# Autodesk Inventor assembly: Z-axis Left Plate
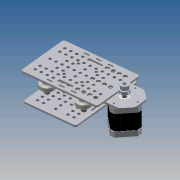
[picture p0: Inventor's stored thumbnail of the model, 180x180]
Saved by Autodesk Inventor 2016 (Build 200138000, 138)
## iProperties
Created: 2015-10-03
Part Number: Z-axis Left Plate
Document SubType Name: Assembly
Designer: Solomon
Author: Solomon
## Documents named in this file (7)
- C:\Users\Solomon\Documents\Inventor\jonathan-printer\Z-axis Right.iam
- C:\Users\Solomon\Documents\Inventor\jonathan-printer\V Slot Part Files\V Slot Plates\Large Build Plate.ipt
- C:\Users\Solomon\Documents\Inventor\jonathan-printer\V Slot Part Files\assembledwheel.iam
- C:\Users\Solomon\Documents\Inventor\jonathan-printer\M1173041- NEMA 17.ipt
- C:\Users\Solomon\Documents\Inventor\jonathan-printer\V Slot Part Files\V Slot Plates\Threaded Rod Plate.ipt
- C:\Users\Solomon\Documents\Inventor\jonathan-printer\Imported Components\GT2_20tooth\GT2_20tooth.ipt
- C:\Users\Solomon\Documents\Inventor\jonathan-printer\V Slot Part Files\V Slot Plates\Metric 8mm ACME Block.ipt
## Components (11 placed, 6 different names)
1. assembledwheel:1 [sub-assembly] — Angle:8, Mate:15, Mate:20, Angle:16
2. assembledwheel:2 [sub-assembly] — Angle:8, Mate:18, Mate:19, Angle:16, Angle:17
3. assembledwheel:3 [sub-assembly] — Angle:9, Mate:14, Mate:16, Mate:17, Angle:17, Angle:18, Angle:20
4. assembledwheel:4 [sub-assembly] — Mate:6, Mate:21, Mate:22, Angle:18, Angle:19
5. Large Build Plate:2 — Mate:6, Angle:9, Angle:14, Angle:15, Mate:16, Mate:17, Mate:18, Mate:20, Mate:21, Angle:21, Angle:22, Mate:23
6. M1173041- NEMA 17:1 — Mate:24, Angle:23, Angle:24, Insert:1
7. Large Build Plate:3 — Angle:14, Angle:15, Mate:14, Mate:15, Mate:19, Mate:22, Angle:19, Angle:20, Angle:26, Angle:27, Angle:28, Angle:29, Mate:25, Mate:26
8. Threaded Rod Plate:1 — Angle:21, Angle:22, Mate:23, Mate:24, Angle:23, Angle:24, Angle:25
9. GT2_20tooth:1 — Angle:25, Insert:1
10. Metric 8mm ACME Block:1 — Angle:26, Angle:27, Angle:28, Angle:29, Mate:25, Flush:1, Flush:2, Angle:30, Angle:31, Angle:32
11. Metric 8mm ACME Block:2 — Flush:1, Flush:2, Angle:30, Angle:31, Angle:32, Mate:26
## Relationships (38: Angle 21, Mate 14, Flush 2, Insert 1)
- Mate:6: assembledwheel:4 ↔ Large Build Plate:2
- Angle:8 (0 deg): assembledwheel:1 ↔ assembledwheel:2
- Angle:9 (0 deg): assembledwheel:3 ↔ Large Build Plate:2
- Angle:14 (0 deg): Large Build Plate:2 ↔ Large Build Plate:3
- Angle:15 (0 deg): Large Build Plate:2 ↔ Large Build Plate:3
- Mate:14: assembledwheel:3 ↔ Large Build Plate:3
- Mate:15: assembledwheel:1 ↔ Large Build Plate:3
- Mate:16: assembledwheel:3 ↔ Large Build Plate:2
- Mate:17: assembledwheel:3 ↔ Large Build Plate:2
- Mate:18: assembledwheel:2 ↔ Large Build Plate:2
- Mate:19: assembledwheel:2 ↔ Large Build Plate:3
- Mate:20: assembledwheel:1 ↔ Large Build Plate:2
- Angle:16 (0 deg): assembledwheel:1 ↔ assembledwheel:2
- Angle:17 (0 deg): assembledwheel:2 ↔ assembledwheel:3
- Mate:21: assembledwheel:4 ↔ Large Build Plate:2
- Mate:22: assembledwheel:4 ↔ Large Build Plate:3
- Angle:18 (0 deg): assembledwheel:3 ↔ assembledwheel:4
- Angle:19 (0 deg): assembledwheel:4 ↔ Large Build Plate:3
- Angle:20 (0 deg): assembledwheel:3 ↔ Large Build Plate:3
- Angle:21 (0 deg): Large Build Plate:2 ↔ Threaded Rod Plate:1
- Angle:22 (0 deg): Large Build Plate:2 ↔ Threaded Rod Plate:1
- Mate:23: Large Build Plate:2 ↔ Threaded Rod Plate:1
- Mate:24: M1173041- NEMA 17:1 ↔ Threaded Rod Plate:1
- Angle:23 (0 deg): M1173041- NEMA 17:1 ↔ Threaded Rod Plate:1
- Angle:24 (45 deg): M1173041- NEMA 17:1 ↔ Threaded Rod Plate:1
- Angle:25 (180 deg): Threaded Rod Plate:1 ↔ GT2_20tooth:1
- Insert:1 (-15 mm): M1173041- NEMA 17:1 ↔ GT2_20tooth:1
- Angle:26 (180 deg): Large Build Plate:3 ↔ Metric 8mm ACME Block:1
- Angle:27 (0 deg): Large Build Plate:3 ↔ Metric 8mm ACME Block:1
- Angle:28 (0 deg): Large Build Plate:3 ↔ Metric 8mm ACME Block:1
- Angle:29 (0 deg): Large Build Plate:3 ↔ Metric 8mm ACME Block:1
- Mate:25: Large Build Plate:3 ↔ Metric 8mm ACME Block:1
- Flush:1: Metric 8mm ACME Block:1 ↔ Metric 8mm ACME Block:2
- Flush:2: Metric 8mm ACME Block:1 ↔ Metric 8mm ACME Block:2
- Angle:30 (0 deg): Metric 8mm ACME Block:1 ↔ Metric 8mm ACME Block:2
- Angle:31 (0 deg): Metric 8mm ACME Block:1 ↔ Metric 8mm ACME Block:2
- Angle:32 (0 deg): Metric 8mm ACME Block:1 ↔ Metric 8mm ACME Block:2
- Mate:26: Large Build Plate:3 ↔ Metric 8mm ACME Block:2
